# Autodesk Inventor assembly: Сборка
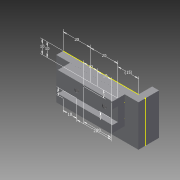
[picture p0: Inventor's stored thumbnail of the model, 180x180]
Saved by Autodesk Inventor 2015 (Build 190159000, 159)
## iProperties
Created: 2016-04-08
Part Number: Сборка
Document SubType Name: Assembly
Designer: Andreas
Author: Andreas
## Documents named in this file (4)
- C:\Users\criit\Desktop\Игры\проект\ласт_ворк_v1.5.2\каретка+деталь к ней\Detal+Karetka.iam
- C:\Users\criit\Desktop\Игры\проект\ласт_ворк_v1.5.2\каретка+деталь к ней\Karetka.ipt
- C:\Users\criit\Desktop\Игры\проект\ласт_ворк_v1.5.2\каретка+деталь к ней\DetalKKaretke.ipt
- C:\Users\criit\Desktop\Игры\проект\ласт_ворк_v1.5.2\каретка+деталь к ней\Сборка\Design Accelerator\Bolted Connection1.iam
## Components (3 placed, 3 different names)
1. Karetka:1 — Rigid:1
2. DetalKKaretke:1 — Rigid:1, Mate:1, Mate:2
3. Bolted Connection:1 [sub-assembly] — Mate:1, Mate:2
## Relationships (3: Mate 2, WeldJoint 1)
- Rigid:1 [WeldJoint]: Karetka:1 ↔ DetalKKaretke:1
- Mate:1: DetalKKaretke:1 ↔ Bolted Connection:1
- Mate:2: DetalKKaretke:1 ↔ Bolted Connection:1
